# Autodesk Inventor assembly: Full Car
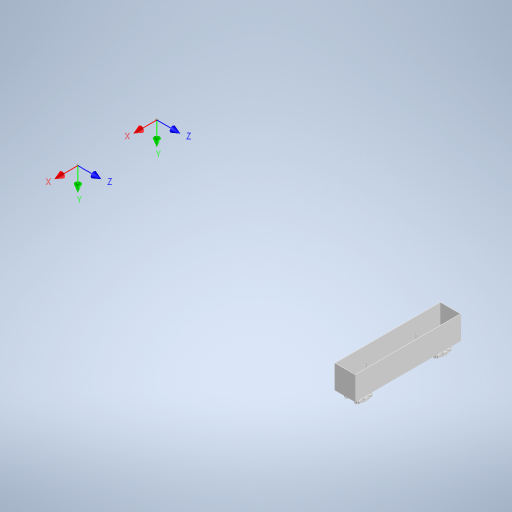
[picture p0: Inventor's stored thumbnail of the model, 512x512]
Saved by Autodesk Inventor 2023 (Build 270158030, 158C)
## iProperties
Created: 2023-02-14
Part Number: Full Car
Document SubType Name: Assembly
Designer: jeremyy
Author: jeremyy
## Documents named in this file (3)
- \\andrew.ad.cmu.edu\users\users1\jeremyy\Documents\Inventor\CMU Bridge\Car\Full Car.iam
- \\andrew.ad.cmu.edu\users\users1\jeremyy\Documents\Inventor\CMU Bridge\Car\Box.ipt
- \\andrew.ad.cmu.edu\users\users1\jeremyy\Documents\Inventor\CMU Bridge\Car\Full Truck.iam
## Components (3 placed, 2 different names)
1. Box:1 — Mate:1, Flush:1, Flush:2, Mate:2, Flush:3, Flush:4
2. Full Truck:1 [sub-assembly] — Mate:1, Flush:1, Flush:2
3. Full Truck:2 [sub-assembly] — Mate:2, Flush:3, Flush:4
## Relationships (6: Flush 4, Mate 2)
- Mate:1: Box:1 ↔ Full Truck:1
- Flush:1: Box:1 ↔ Full Truck:1
- Flush:2: Box:1 ↔ Full Truck:1
- Mate:2: Box:1 ↔ Full Truck:2
- Flush:3: Box:1 ↔ Full Truck:2
- Flush:4: Box:1 ↔ Full Truck:2
